# Autodesk Inventor assembly: ASSEMBLY_Regolith_Container
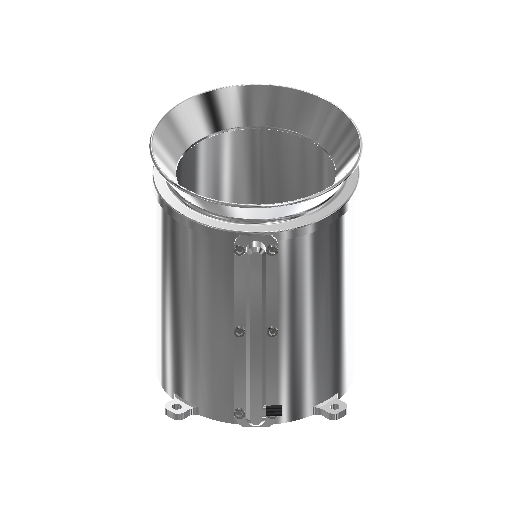
[picture p0: Inventor's stored thumbnail of the model, 512x512]
Saved by Autodesk Inventor 2025 (Build 290162010, 162A)
## iProperties
Created: 2018-09-17
Part Number: ASSEMBLY_Regolith_Container
Document SubType Name: Assembly
Designer: Andrzej
Mass: 44.0999 g
Surface Area: 294.127 cm^2
Volume: 16.2231 cm^3
Density: 2.71833 g/cm^3
Author: Andrzej
## Documents named in this file (6)
- D:\_ANDRZEJ_LACZEWSKI\_OTHER\MECH - My entry for the NASA Lunar Sampling System Design Challenge\MCAD\1_REV1\ASSEMBLY_MAIN_REVA\ASSEMBLY_Regolith_Container.iam
- D:\_ANDRZEJ_LACZEWSKI\_OTHER\MECH - My entry for the NASA Lunar Sampling System Design Challenge\MCAD\1_REV1\ASSEMBLY_MAIN_REVA\ASSEMBLY_Regolith_container_level_sensor.ipt
- D:\_ANDRZEJ_LACZEWSKI\_OTHER\MECH - My entry for the NASA Lunar Sampling System Design Challenge\MCAD\1_REV1\ASSEMBLY_MAIN_REVA\CNCM_ALU_Regolith_container.ipt
- D:\_ANDRZEJ_LACZEWSKI\_OTHER\MECH - My entry for the NASA Lunar Sampling System Design Challenge\MCAD\1_REV1\ASSEMBLY_MAIN_REVA\CNCM_ALU_Regolith_container_funnel.ipt
- D:\_ANDRZEJ_LACZEWSKI\_OTHER\MECH - My entry for the NASA Lunar Sampling System Design Challenge\MCAD\1_REV1\ASSEMBLY_MAIN_REVA\CNCT_STEEL_M1,6x2_Screw.ipt
- D:\_ANDRZEJ_LACZEWSKI\_OTHER\MECH - My entry for the NASA Lunar Sampling System Design Challenge\MCAD\1_REV1\ASSEMBLY_MAIN_REVA\OTH_15mm_rock.ipt
## Components (16 placed, 5 different names)
1. ASSEMBLY_Regolith_container_level_sensor:1 — Mate:1, Mate:2, Flush:1, Mate:5, Mate:6, Mate:7, Mate:8, Mate:9, Mate:10, Mate:11, Mate:12, Mate:13, Mate:14, Mate:15, Mate:16
2. CNCM_ALU_Regolith_container:1 — Mate:1, Mate:2, Flush:1, Mate:3, Mate:4
3. CNCM_ALU_Regolith_container_funnel:1 — Mate:3, Mate:4
4. CNCT_STEEL_M1,6x2_Screw:1 — Mate:8, Mate:14
5. CNCT_STEEL_M1,6x2_Screw:2 — Mate:6, Mate:12
6. CNCT_STEEL_M1,6x2_Screw:3 — Mate:7, Mate:13
7. CNCT_STEEL_M1,6x2_Screw:4 — Mate:5, Mate:11
8. CNCT_STEEL_M1,6x2_Screw:5 — Mate:10, Mate:15
9. CNCT_STEEL_M1,6x2_Screw:6 — Mate:9, Mate:16
10. OTH_15mm_rock:1
11. OTH_15mm_rock:2
12. OTH_15mm_rock:3
13. OTH_15mm_rock:4
14. OTH_15mm_rock:5
15. OTH_15mm_rock:6
16. OTH_15mm_rock:7
## Relationships (17: Mate 16, Flush 1)
- Mate:1: ASSEMBLY_Regolith_container_level_sensor:1 ↔ CNCM_ALU_Regolith_container:1
- Mate:2: ASSEMBLY_Regolith_container_level_sensor:1 ↔ CNCM_ALU_Regolith_container:1
- Flush:1: ASSEMBLY_Regolith_container_level_sensor:1 ↔ CNCM_ALU_Regolith_container:1
- Mate:3: CNCM_ALU_Regolith_container:1 ↔ CNCM_ALU_Regolith_container_funnel:1
- Mate:4: CNCM_ALU_Regolith_container:1 ↔ CNCM_ALU_Regolith_container_funnel:1
- Mate:5: ASSEMBLY_Regolith_container_level_sensor:1 ↔ CNCT_STEEL_M1,6x2_Screw:4
- Mate:6: ASSEMBLY_Regolith_container_level_sensor:1 ↔ CNCT_STEEL_M1,6x2_Screw:2
- Mate:7: ASSEMBLY_Regolith_container_level_sensor:1 ↔ CNCT_STEEL_M1,6x2_Screw:3
- Mate:8: ASSEMBLY_Regolith_container_level_sensor:1 ↔ CNCT_STEEL_M1,6x2_Screw:1
- Mate:9: ASSEMBLY_Regolith_container_level_sensor:1 ↔ CNCT_STEEL_M1,6x2_Screw:6
- Mate:10: ASSEMBLY_Regolith_container_level_sensor:1 ↔ CNCT_STEEL_M1,6x2_Screw:5
- Mate:11: ASSEMBLY_Regolith_container_level_sensor:1 ↔ CNCT_STEEL_M1,6x2_Screw:4
- Mate:12: ASSEMBLY_Regolith_container_level_sensor:1 ↔ CNCT_STEEL_M1,6x2_Screw:2
- Mate:13: ASSEMBLY_Regolith_container_level_sensor:1 ↔ CNCT_STEEL_M1,6x2_Screw:3
- Mate:14: ASSEMBLY_Regolith_container_level_sensor:1 ↔ CNCT_STEEL_M1,6x2_Screw:1
- Mate:15: ASSEMBLY_Regolith_container_level_sensor:1 ↔ CNCT_STEEL_M1,6x2_Screw:5
- Mate:16: ASSEMBLY_Regolith_container_level_sensor:1 ↔ CNCT_STEEL_M1,6x2_Screw:6
